# Autodesk Inventor assembly: катушка+мотор
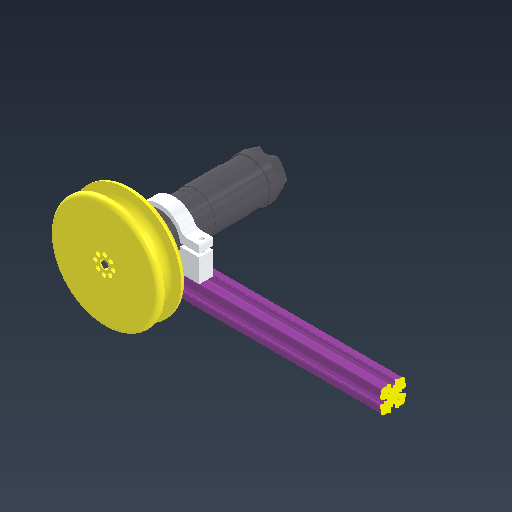
[picture p0: Inventor's stored thumbnail of the model, 512x512]
Saved by Autodesk Inventor 2025 (Build 290162000, 162)
## iProperties
Created: 2025-01-28
Part Number: катушка+мотор
Document SubType Name: Assembly
Designer: GameHD
Author: GameHD
## Documents named in this file (6)
- C:\Users\GameHD\Desktop\phantom 16950\катушка+мотор.iam
- C:\Users\GameHD\Desktop\phantom 16950\профиль каркас ГОРИЗОНТ пенпер.ipt
- C:\Users\GameHD\Desktop\phantom 16950\katushechka_pushechka\katushechka_pushechka.ipt
- C:\Users\GameHD\Desktop\phantom 16950\katushechka_pushechka 2\katushechka_pushechka 2.ipt
- C:\Users\GameHD\Desktop\phantom 16950\39089_txm-motormount\39089_txm-motormount.ipt
- C:\Users\GameHD\Desktop\phantom 16950\REV-41-1211\REV-41-1211.ipt
## Components (5 placed, 5 different names)
1. профиль каркас ГОРИЗОНТ пенпер:1
2. katushechka_pushechka:1
3. katushechka_pushechka 2:1
4. 39089_txm-motormount:1
5. REV-41-1211:1
## Relationships (7: Mate 5, Flush 2)
- [Mate]: katushechka_pushechka:1 ↔ katushechka_pushechka 2:1
- [Mate]: katushechka_pushechka:1 ↔ katushechka_pushechka 2:1
- [Mate]: профиль каркас ГОРИЗОНТ пенпер:1 ↔ 39089_txm-motormount:1
- [Flush]: профиль каркас ГОРИЗОНТ пенпер:1 ↔ 39089_txm-motormount:1
- [Mate]: 39089_txm-motormount:1 ↔ REV-41-1211:1
- [Mate]: katushechka_pushechka 2:1 ↔ REV-41-1211:1
- [Flush]: katushechka_pushechka 2:1 ↔ REV-41-1211:1
